# Autodesk Inventor assembly: sisaku syasyutu
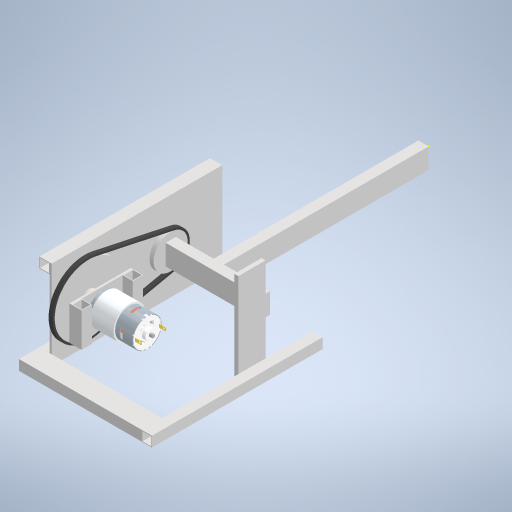
[picture p0: Inventor's stored thumbnail of the model, 512x512]
Saved by Autodesk Inventor 2023 (Build 270158000, 158)
## iProperties
Created: 2022-04-19
Part Number: sisaku syasyutu
Document SubType Name: Assembly
Designer: yuta
Author: yuta
## Documents named in this file (13)
- C:\Users\yuta\Documents\NHK\sisaku syasyutu.iam
- C:\Users\yuta\Documents\NHK\NHK_t0_3.ipt
- C:\Users\yuta\Documents\NHK\RS775_CAD_IAM\モーター RS775-8513DF.iam
- C:\Users\yuta\Documents\NHK\NHK_t0_4.ipt
- C:\Users\yuta\Documents\NHK\NHK_t0_5.ipt
- C:\Users\yuta\Documents\NHK\NHK_t0_6.ipt
- C:\Users\yuta\Documents\NHK\NHK_t0_7.ipt
- C:\Users\yuta\Documents\NHK\NHK_t0_8.ipt
- C:\Users\yuta\Documents\NHK\NHK_t0_9.ipt
- C:\Users\yuta\Documents\NHK\NHK_t0_11.ipt
- C:\Users\yuta\Documents\NHK\NHK_t0_12.ipt
- C:\Users\yuta\Documents\NHK\NHK_t0_13.ipt
- C:\Users\yuta\Documents\NHK\NHK_t0_14.ipt
## Components (16 placed, 12 different names)
1. NHK_t0_3:1 — メイト:3, フラッシュ:1, メイト:7, メイト:8, メイト:9, メイト:10
2. NHK_t0_4:1 — メイト:3, フラッシュ:1, メイト:4, フラッシュ:2
3. NHK_t0_5:1 — メイト:4, フラッシュ:2, メイト:5, フラッシュ:3, メイト:6
4. NHK_t0_6:1 — メイト:5, フラッシュ:3, メイト:6
5. NHK_t0_7:1 — メイト:7, メイト:8, メイト:13
6. NHK_t0_7:2 — メイト:9, メイト:10, メイト:16, メイト:17
7. モーター RS775-8513DF:1 [sub-assembly] — メイト:11, メイト:12, メイト:13
8. NHK_t0_8:1 — メイト:11, メイト:12, メイト:14, フラッシュ:4, フラッシュ:5, メイト:15, フラッシュ:6, フラッシュ:7
9. NHK_t0_9:1 — メイト:14, フラッシュ:4, フラッシュ:5
10. NHK_t0_9:2 — メイト:15, フラッシュ:6, フラッシュ:7
11. NHK_t0_11:1 — メイト:16, メイト:17, フラッシュ:8, メイト:18, フラッシュ:9, メイト:19, フラッシュ:10, フラッシュ:11
12. NHK_t0_12:1 — フラッシュ:8, メイト:18, フラッシュ:9
13. NHK_t0_12:2 — メイト:19, フラッシュ:10, フラッシュ:11, メイト:20, フラッシュ:12, フラッシュ:13
14. NHK_t0_13:1 — メイト:20, フラッシュ:12, フラッシュ:13, メイト:21, フラッシュ:14, フラッシュ:15
15. NHK_t0_12:3 — メイト:21, フラッシュ:14, フラッシュ:15
16. NHK_t0_14:1
## Relationships (34: Mate 19, Flush 15)
- メイト:3 [Mate]: NHK_t0_3:1 ↔ NHK_t0_4:1
- フラッシュ:1 [Flush]: NHK_t0_3:1 ↔ NHK_t0_4:1
- メイト:4 [Mate]: NHK_t0_4:1 ↔ NHK_t0_5:1
- フラッシュ:2 [Flush]: NHK_t0_4:1 ↔ NHK_t0_5:1
- メイト:5 [Mate]: NHK_t0_5:1 ↔ NHK_t0_6:1
- フラッシュ:3 [Flush]: NHK_t0_5:1 ↔ NHK_t0_6:1
- メイト:6 [Mate] (67.5 mm): NHK_t0_5:1 ↔ NHK_t0_6:1
- メイト:7 [Mate]: NHK_t0_3:1 ↔ NHK_t0_7:1
- メイト:8 [Mate]: NHK_t0_3:1 ↔ NHK_t0_7:1
- メイト:9 [Mate]: NHK_t0_3:1 ↔ NHK_t0_7:2
- メイト:10 [Mate]: NHK_t0_3:1 ↔ NHK_t0_7:2
- メイト:11 [Mate]: モーター RS775-8513DF:1 ↔ NHK_t0_8:1
- メイト:12 [Mate]: モーター RS775-8513DF:1 ↔ NHK_t0_8:1
- メイト:13 [Mate]: NHK_t0_7:1 ↔ モーター RS775-8513DF:1
- メイト:14 [Mate]: NHK_t0_8:1 ↔ NHK_t0_9:1
- フラッシュ:4 [Flush]: NHK_t0_8:1 ↔ NHK_t0_9:1
- フラッシュ:5 [Flush]: NHK_t0_8:1 ↔ NHK_t0_9:1
- メイト:15 [Mate]: NHK_t0_8:1 ↔ NHK_t0_9:2
- フラッシュ:6 [Flush]: NHK_t0_8:1 ↔ NHK_t0_9:2
- フラッシュ:7 [Flush]: NHK_t0_8:1 ↔ NHK_t0_9:2
- メイト:16 [Mate]: NHK_t0_7:2 ↔ NHK_t0_11:1
- メイト:17 [Mate]: NHK_t0_7:2 ↔ NHK_t0_11:1
- フラッシュ:8 [Flush]: NHK_t0_11:1 ↔ NHK_t0_12:1
- メイト:18 [Mate]: NHK_t0_11:1 ↔ NHK_t0_12:1
- フラッシュ:9 [Flush]: NHK_t0_11:1 ↔ NHK_t0_12:1
- メイト:19 [Mate]: NHK_t0_11:1 ↔ NHK_t0_12:2
- フラッシュ:10 [Flush]: NHK_t0_11:1 ↔ NHK_t0_12:2
- フラッシュ:11 [Flush]: NHK_t0_11:1 ↔ NHK_t0_12:2
- メイト:20 [Mate]: NHK_t0_12:2 ↔ NHK_t0_13:1
- フラッシュ:12 [Flush]: NHK_t0_12:2 ↔ NHK_t0_13:1
- フラッシュ:13 [Flush]: NHK_t0_12:2 ↔ NHK_t0_13:1
- メイト:21 [Mate]: NHK_t0_13:1 ↔ NHK_t0_12:3
- フラッシュ:14 [Flush]: NHK_t0_13:1 ↔ NHK_t0_12:3
- フラッシュ:15 [Flush]: NHK_t0_13:1 ↔ NHK_t0_12:3
